# Autodesk Inventor assembly: A2017_T4_12
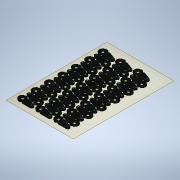
[picture p0: Inventor's stored thumbnail of the model, 180x180]
Saved by Autodesk Inventor 2020 (Build 240168000, 168)
## iProperties
Created: 2021-08-27
Part Number: A2017_T4_12
Document SubType Name: Assembly
Designer: Masato
Author: Masato
## Documents named in this file (3)
- D:\GitHub\inventor\SUSTAINA-OP\Cam\A2017_T4_12.iam
- D:\GitHub\inventor\SUSTAINA-OP\Cam\DisposableBoard.ipt
- D:\GitHub\inventor\SUSTAINA-OP\LowerBody\Ankle\Ankle_side_pitch_frame.ipt
## Components (40 placed, 2 different names)
1. DisposableBoard:1 — メイト:2, メイト:1, フラッシュ:1, フラッシュ:2, メイト:4, フラッシュ:3, 正接:1, メイト:5, 正接:2, メイト:9, 正接:3, メイト:11, メイト:12
2. Ankle_side_pitch_frame:37 — メイト:9, 正接:3, メイト:10, 正接:4
3. Ankle_side_pitch_frame:38 — メイト:11, メイト:13, 正接:4, 正接:5
4. Ankle_side_pitch_frame:39 — メイト:12, メイト:14, 正接:5
5. Ankle_side_pitch_frame:1 — メイト:4, フラッシュ:3, 正接:1, メイト:6
6. Ankle_side_pitch_frame:2 — メイト:5, メイト:6, 正接:2
7. Ankle_side_pitch_frame:3
8. Ankle_side_pitch_frame:4
9. Ankle_side_pitch_frame:5
10. Ankle_side_pitch_frame:6
11. Ankle_side_pitch_frame:7
12. Ankle_side_pitch_frame:8
13. Ankle_side_pitch_frame:9
14. Ankle_side_pitch_frame:10
15. Ankle_side_pitch_frame:11
16. Ankle_side_pitch_frame:12
17. Ankle_side_pitch_frame:13
18. Ankle_side_pitch_frame:14
19. Ankle_side_pitch_frame:15
20. Ankle_side_pitch_frame:16
21. Ankle_side_pitch_frame:17
22. Ankle_side_pitch_frame:18
23. Ankle_side_pitch_frame:19
24. Ankle_side_pitch_frame:20
25. Ankle_side_pitch_frame:21
26. Ankle_side_pitch_frame:22
27. Ankle_side_pitch_frame:23
28. Ankle_side_pitch_frame:24
29. Ankle_side_pitch_frame:25
30. Ankle_side_pitch_frame:26
31. Ankle_side_pitch_frame:27
32. Ankle_side_pitch_frame:28
33. Ankle_side_pitch_frame:29
34. Ankle_side_pitch_frame:30
35. Ankle_side_pitch_frame:31
36. Ankle_side_pitch_frame:32 — メイト:10
37. Ankle_side_pitch_frame:33
38. Ankle_side_pitch_frame:34 — メイト:13
39. Ankle_side_pitch_frame:35
40. Ankle_side_pitch_frame:36 — メイト:14
## Component patterns: (18 elements, first: Ankle_side_pitch_frame:1 + Ankle_side_pitch_frame:2)
## Relationships (19: Mate 11, Tangent 5, Flush 3)
- メイト:2 [Mate]: DisposableBoard:1
- メイト:1 [Mate]: DisposableBoard:1
- フラッシュ:1 [Flush]: DisposableBoard:1
- フラッシュ:2 [Flush]: DisposableBoard:1
- メイト:4 [Mate]: DisposableBoard:1 ↔ Ankle_side_pitch_frame:1
- フラッシュ:3 [Flush] (2 mm): DisposableBoard:1 ↔ Ankle_side_pitch_frame:1
- 正接:1 [Tangent] (2 mm): DisposableBoard:1 ↔ Ankle_side_pitch_frame:1
- メイト:5 [Mate]: DisposableBoard:1 ↔ Ankle_side_pitch_frame:2
- メイト:6 [Mate] (2.5 mm): Ankle_side_pitch_frame:1 ↔ Ankle_side_pitch_frame:2
- 正接:2 [Tangent] (8 mm): DisposableBoard:1 ↔ Ankle_side_pitch_frame:2
- メイト:9 [Mate]: DisposableBoard:1 ↔ Ankle_side_pitch_frame:37
- 正接:3 [Tangent] (2 mm): DisposableBoard:1 ↔ Ankle_side_pitch_frame:37
- メイト:10 [Mate] (2.5 mm): Ankle_side_pitch_frame:37 ↔ Ankle_side_pitch_frame:32
- メイト:11 [Mate]: DisposableBoard:1 ↔ Ankle_side_pitch_frame:38
- メイト:12 [Mate]: DisposableBoard:1 ↔ Ankle_side_pitch_frame:39
- メイト:13 [Mate] (2.5 mm): Ankle_side_pitch_frame:38 ↔ Ankle_side_pitch_frame:34
- メイト:14 [Mate] (2.5 mm): Ankle_side_pitch_frame:39 ↔ Ankle_side_pitch_frame:36
- 正接:4 [Tangent] (2.5 mm): Ankle_side_pitch_frame:37 ↔ Ankle_side_pitch_frame:38
- 正接:5 [Tangent] (2.5 mm): Ankle_side_pitch_frame:38 ↔ Ankle_side_pitch_frame:39
